# Autodesk Inventor assembly: collector rotator assembly
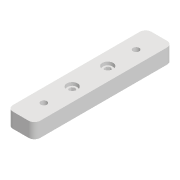
[picture p0: Inventor's stored thumbnail of the model, 180x180]
Saved by Autodesk Inventor 2020 (Build 240168000, 168)
## iProperties
Created: 2019-11-06
Part Number: collector rotator assembly
Document SubType Name: Assembly
Designer: ball
Author: ball
## Documents named in this file (3)
- C:\FTC\FTC8863CAD\2019 Robot\Collection\collector rotator assembly.iam
- C:\FTC\FTC8863CAD\2019 Robot\Collection\Collection rotation adapter.ipt
- C:\FTC\FTC8863CAD\2019 Robot\Collection\6-32x5-16.ipt
## Components (3 placed, 2 different names)
1. Collection rotation adapter:1 — Mate:1, Mate:2, Mate:3, Mate:4
2. 6-32x5-16:1 — Mate:3, Mate:4
3. 6-32x5-16:2 — Mate:1, Mate:2
## Relationships (4: Mate 4)
- Mate:1: Collection rotation adapter:1 ↔ 6-32x5-16:2
- Mate:2: Collection rotation adapter:1 ↔ 6-32x5-16:2
- Mate:3: Collection rotation adapter:1 ↔ 6-32x5-16:1
- Mate:4: Collection rotation adapter:1 ↔ 6-32x5-16:1
